# Autodesk Inventor assembly: Extension Board Assembly
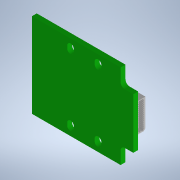
[picture p0: Inventor's stored thumbnail of the model, 180x180]
Saved by Autodesk Inventor 2021 (Build 250183000, 183)
## iProperties
Created: 2020-04-20
Part Number: Extension Board Assembly
Document SubType Name: Assembly
Designer: jgray
Author: jgray
## Documents named in this file (3)
- M:\Printed Electronics\Gas Sensors\Prototypes\Prototype II -Cartridge Reader V3\Extension Board Assembly.iam
- M:\Printed Electronics\Gas Sensors\Prototypes\Prototype II -Cartridge Reader V3\533093070.ipt
- M:\Printed Electronics\Gas Sensors\Prototypes\Prototype II -Cartridge Reader V3\Extension PCB.ipt
## Components (2 placed, 2 different names)
1. 533093070:1 — Mate:1, Angle:1, Mate:2, Mate:3
2. Extension PCB:1 — Mate:1, Angle:1, Mate:2, Mate:3
## Relationships (4: Mate 3, Angle 1)
- Mate:1: 533093070:1 ↔ Extension PCB:1
- Angle:1 (0 deg): 533093070:1 ↔ Extension PCB:1
- Mate:2: 533093070:1 ↔ Extension PCB:1
- Mate:3 (0.09 mm): 533093070:1 ↔ Extension PCB:1
